# Autodesk Inventor assembly: Assembly_Trial_3
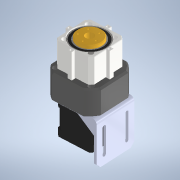
[picture p0: Inventor's stored thumbnail of the model, 180x180]
Saved by Autodesk Inventor 2022 (Build 260153000, 153)
## iProperties
Created: 2022-01-15
Part Number: Assembly_Trial_3
Document SubType Name: Assembly
Designer: Mlees
Author: Mlees
## Documents named in this file (19)
- F:\404 Engineering Arm\Assembly_Trial_3.iam
- F:\404 Engineering Arm\Downloaded Parts\nema17-speed-reducer-1.snapshot.9\24_Teeth_Sun_Gear.step.ipt
- F:\404 Engineering Arm\Downloaded Parts\nema17-speed-reducer-1.snapshot.9\36_Teeth_Planet_Gear.step.ipt
- F:\404 Engineering Arm\Downloaded Parts\nema17-speed-reducer-1.snapshot.9\96_Teeth_Gear.step.ipt
- F:\404 Engineering Arm\Downloaded Parts\nema17-speed-reducer-1.snapshot.9\Gear_Cover.ipt
- F:\404 Engineering Arm\Downloaded Parts\nema17-speed-reducer-1.snapshot.9\Plamet_Carrier.ipt
- F:\404 Engineering Arm\Downloaded Parts\90751A113_18-8 Stainless Steel Socket Head Screws.ipt
- F:\404 Engineering Arm\Downloaded Parts\91292A022_18-8 Stainless Steel Socket Head Screw.ipt
- F:\404 Engineering Arm\Downloaded Parts\90592A085_Steel Hex Nut.ipt
- F:\404 Engineering Arm\Downloaded Parts\nema-17-motor-mount-1.snapshot.1\NEMA_17_Bracket.ipt
- F:\404 Engineering Arm\Downloaded Parts\nema17-speed-reducer-1.snapshot.9\Thread Insert M3 x 6mm v2.step.iam
- F:\404 Engineering Arm\Downloaded Parts\Harmonic_Drive\Nema 17.ipt
- F:\404 Engineering Arm\Downloaded Parts\Harmonic_Drive\91290A144_BLACK-OXIDE CLASS 12.9 SOCKET HEAD CAP SCREW v1 v1.ipt
- F:\404 Engineering Arm\Downloaded Parts\Harmonic_Drive\Bearing.ipt
- F:\404 Engineering Arm\Downloaded Parts\Harmonic_Drive\Big Bearing v1.ipt
- F:\404 Engineering Arm\Downloaded Parts\Harmonic_Drive\Bigger_Bearing.ipt
- F:\404 Engineering Arm\Downloaded Parts\Harmonic_Drive\Harmonic_Drive_STEP_Cover v2.ipt
- F:\404 Engineering Arm\Downloaded Parts\Harmonic_Drive\Harmonic_Drive_STEP_Gear_TPU v2.ipt
- F:\404 Engineering Arm\Downloaded Parts\Harmonic_Drive\Harmonic_Drive_STEP_Spinner v1.ipt
## Components (33 placed, 18 different names)
1. 24_Teeth_Sun_Gear.step:1 — Rotational:6
2. 36_Teeth_Planet_Gear.step:1 — Rotational:3
3. 96_Teeth_Gear.step:1 — Rigid:2, Rigid:3, Rigid:4, Rigid:5, Rotational:7, Rotational:8, Rotational:9, Rotational:10, Rigid:7
4. Gear_Cover:1 — Rigid:7, Rigid:8, Rigid:9, Rigid:10, Rigid:11, Rigid:13
5. Plamet_Carrier:1 — Rotational:1, Rotational:3, Rotational:4, Rotational:5, Rotational:6
6. 90751A113_18-8 Stainless Steel Socket Head Screws:1 — Rigid:3
7. 90751A113_18-8 Stainless Steel Socket Head Screws:2 — Rigid:4
8. 90751A113_18-8 Stainless Steel Socket Head Screws:3 — Rigid:5
9. 91292A022_18-8 Stainless Steel Socket Head Screw:1 — Rotational:1, Rigid:6
10. 90592A085_Steel Hex Nut:2 — Rigid:6, Rotational:11
11. NEMA_17_Bracket:1 — Rigid:2, Rigid:12
12. 36_Teeth_Planet_Gear.step:2 — Rotational:4
13. 36_Teeth_Planet_Gear.step:4 — Rotational:5
14. Thread Insert M3 x 6mm v2.step:1 [sub-assembly] — Rotational:7
15. Thread Insert M3 x 6mm v2.step:2 [sub-assembly] — Rotational:8
16. Thread Insert M3 x 6mm v2.step:3 [sub-assembly] — Rotational:9
17. Thread Insert M3 x 6mm v2.step:4 [sub-assembly] — Rotational:10
18. 90751A113_18-8 Stainless Steel Socket Head Screws:4 — Rigid:8
19. 90751A113_18-8 Stainless Steel Socket Head Screws:5 — Rigid:9
20. 90751A113_18-8 Stainless Steel Socket Head Screws:6 — Rigid:10
21. 90751A113_18-8 Stainless Steel Socket Head Screws:7 — Rigid:11
22. 90592A085_Steel Hex Nut:3 — Rotational:11, Rotational:12
23. 90592A085_Steel Hex Nut:4 — Rotational:12, Rigid:14
24. Nema 17:1 — Rigid:12
25. 91290A144_BLACK-OXIDE CLASS 12.9 SOCKET HEAD CAP SCREW v1 v1:1 — Rotational:13
26. Bearing:1 — Rigid:15, Rotational:13
27. Big Bearing v1:1 — Rotational:17
28. Bigger_Bearing:1 — Rotational:15, Rotational:16
29. Harmonic_Drive_STEP_Cover v2:1 — Rigid:13, Rotational:17
30. Harmonic_Drive_STEP_Gear_TPU v2:1 — Rotational:16
31. Harmonic_Drive_STEP_Spinner v1:1 — Rigid:14, Rigid:15, Rigid:16, Rotational:15
32. Bearing:2 — Rigid:16, Rotational:14
33. 91290A144_BLACK-OXIDE CLASS 12.9 SOCKET HEAD CAP SCREW v1 v1:2 — Rotational:14
## Relationships (31: RevoluteJoint 16, WeldJoint 15)
- Rigid:2 [WeldJoint]: 96_Teeth_Gear.step:1 ↔ NEMA_17_Bracket:1
- Rigid:3 [WeldJoint]: 96_Teeth_Gear.step:1 ↔ 90751A113_18-8 Stainless Steel Socket Head Screws:1
- Rigid:4 [WeldJoint]: 96_Teeth_Gear.step:1 ↔ 90751A113_18-8 Stainless Steel Socket Head Screws:2
- Rigid:5 [WeldJoint]: 96_Teeth_Gear.step:1 ↔ 90751A113_18-8 Stainless Steel Socket Head Screws:3
- Rotational:1 [RevoluteJoint]: Plamet_Carrier:1 ↔ 91292A022_18-8 Stainless Steel Socket Head Screw:1
- Rotational:3 [RevoluteJoint]: 36_Teeth_Planet_Gear.step:1 ↔ Plamet_Carrier:1
- Rotational:4 [RevoluteJoint]: Plamet_Carrier:1 ↔ 36_Teeth_Planet_Gear.step:2
- Rotational:5 [RevoluteJoint]: Plamet_Carrier:1 ↔ 36_Teeth_Planet_Gear.step:4
- Rotational:6 [RevoluteJoint]: 24_Teeth_Sun_Gear.step:1 ↔ Plamet_Carrier:1
- Rigid:6 [WeldJoint] (-2 mm): 91292A022_18-8 Stainless Steel Socket Head Screw:1 ↔ 90592A085_Steel Hex Nut:2
- Rotational:7 [RevoluteJoint]: 96_Teeth_Gear.step:1 ↔ Thread Insert M3 x 6mm v2.step:1
- Rotational:8 [RevoluteJoint]: 96_Teeth_Gear.step:1 ↔ Thread Insert M3 x 6mm v2.step:2
- Rotational:9 [RevoluteJoint]: 96_Teeth_Gear.step:1 ↔ Thread Insert M3 x 6mm v2.step:3
- Rotational:10 [RevoluteJoint]: 96_Teeth_Gear.step:1 ↔ Thread Insert M3 x 6mm v2.step:4
- Rigid:7 [WeldJoint]: 96_Teeth_Gear.step:1 ↔ Gear_Cover:1
- Rigid:8 [WeldJoint]: Gear_Cover:1 ↔ 90751A113_18-8 Stainless Steel Socket Head Screws:4
- Rigid:9 [WeldJoint]: Gear_Cover:1 ↔ 90751A113_18-8 Stainless Steel Socket Head Screws:5
- Rigid:10 [WeldJoint]: Gear_Cover:1 ↔ 90751A113_18-8 Stainless Steel Socket Head Screws:6
- Rigid:11 [WeldJoint]: Gear_Cover:1 ↔ 90751A113_18-8 Stainless Steel Socket Head Screws:7
- Rotational:11 [RevoluteJoint]: 90592A085_Steel Hex Nut:2 ↔ 90592A085_Steel Hex Nut:3
- Rotational:12 [RevoluteJoint]: 90592A085_Steel Hex Nut:3 ↔ 90592A085_Steel Hex Nut:4
- Rigid:12 [WeldJoint]: NEMA_17_Bracket:1 ↔ Nema 17:1
- Rigid:13 [WeldJoint]: Gear_Cover:1 ↔ Harmonic_Drive_STEP_Cover v2:1
- Rigid:14 [WeldJoint]: 90592A085_Steel Hex Nut:4 ↔ Harmonic_Drive_STEP_Spinner v1:1
- Rigid:15 [WeldJoint]: Bearing:1 ↔ Harmonic_Drive_STEP_Spinner v1:1
- Rigid:16 [WeldJoint]: Harmonic_Drive_STEP_Spinner v1:1 ↔ Bearing:2
- Rotational:13 [RevoluteJoint]: 91290A144_BLACK-OXIDE CLASS 12.9 SOCKET HEAD CAP SCREW v1 v1:1 ↔ Bearing:1
- Rotational:14 [RevoluteJoint]: Bearing:2 ↔ 91290A144_BLACK-OXIDE CLASS 12.9 SOCKET HEAD CAP SCREW v1 v1:2
- Rotational:15 [RevoluteJoint]: Bigger_Bearing:1 ↔ Harmonic_Drive_STEP_Spinner v1:1
- Rotational:16 [RevoluteJoint]: Bigger_Bearing:1 ↔ Harmonic_Drive_STEP_Gear_TPU v2:1
- Rotational:17 [RevoluteJoint]: Big Bearing v1:1 ↔ Harmonic_Drive_STEP_Cover v2:1
